# Autodesk Inventor assembly: B Drive
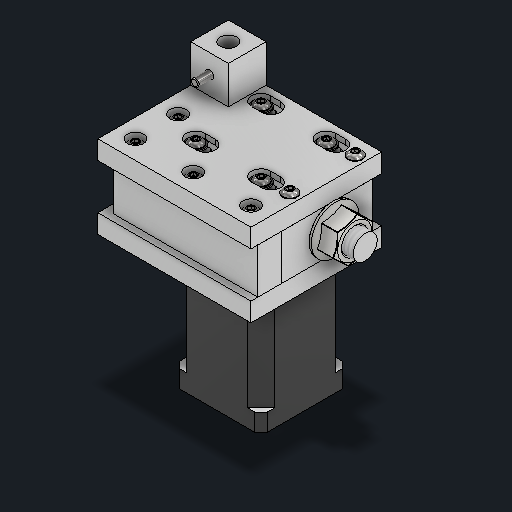
[picture p0: Inventor's stored thumbnail of the model, 512x512]
Saved by Autodesk Inventor 2025.1 (Build 291241020, 241B)
## iProperties
Created: 2025-05-09
Part Number: B Drive
Document SubType Name: Assembly
Designer: AdminForWorker
Title: B Drive
Author: AdminForWorker
## Documents named in this file (10)
- C:\Users\Joshua Eah\Documents\Voron 0.2\CAD\Master Assembly\Motion\AB Drives\Drives\B Drive.iam
- C:\Users\Joshua Eah\Documents\Voron 0.2\CAD\Machined Parts\AB Drives\B Drive\B Drive Assembly.iam
- C:\Users\Joshua Eah\Documents\Voron 0.2\CAD\Master Assembly\Hardware\M3x10 BHCS.ipt
- C:\Users\Joshua Eah\Documents\Voron 0.2\CAD\Master Assembly\Hardware\M3x35 BHCS.ipt
- C:\Users\Joshua Eah\Documents\Voron 0.2\CAD\Master Assembly\Hardware\M3x30 BHCS.ipt
- C:\Users\Joshua Eah\Documents\Voron 0.2\CAD\Master Assembly\Hardware\F623 Stack.iam
- C:\Users\Joshua Eah\Documents\Voron 0.2\CAD\Master Assembly\Hardware\M3 Hexnut.ipt
- C:\Users\Joshua Eah\Documents\Voron 0.2\CAD\Master Assembly\Hardware\M3_Washer.ipt
- C:\Users\Joshua Eah\Documents\Voron 0.2\CAD\Master Assembly\Motion\AB Drives\Motor Assembly\GT2 20T 6mm Pulley.iam
- C:\Users\Joshua Eah\Documents\Voron 0.2\CAD\Master Assembly\Motion\AB Drives\Motor Assembly\Nema14.ipt
## Components (26 placed, 9 different names)
1. B Drive Assembly:1 [sub-assembly] — Insert:4, Insert:5, Insert:10, Insert:11, Insert:12, Insert:13, Mate:5
2. GT2 20T 6mm Pulley:1 [sub-assembly] — Mate:1, Mate:2
3. Nema14:1 — Mate:1, Mate:2, Mate:3, Mate:4, Mate:5
4. M3x10 BHCS:1
5. M3x35 BHCS:1 — Insert:9, Mate:3
6. M3x35 BHCS:2
7. M3x35 BHCS:3
8. M3x35 BHCS:4
9. M3x35 BHCS:5 — Insert:7, Mate:4
10. M3x35 BHCS:6
11. M3x35 BHCS:7 — Insert:8
12. M3x35 BHCS:8 — Insert:6
13. M3x35 BHCS:9 — Insert:3, Insert:4
14. M3x30 BHCS:1
15. M3x30 BHCS:2 — Insert:5
16. M3 Hexnut:1
17. M3 Hexnut:2
18. M3 Hexnut:3
19. M3 Hexnut:4 — Insert:3
20. M3 Washer:1 — Insert:9, Insert:12
21. M3 Washer:2 — Insert:6, Insert:11
22. M3 Washer:3 — Insert:8, Insert:13
23. M3 Washer:4 — Insert:7, Insert:10
24. F623 Stack:1 [sub-assembly]
25. F623 Stack:2 [sub-assembly]
26. F623 Stack:3 [sub-assembly]
## Relationships (18: Insert 13, Mate 5)
- [Insert]: B Drive Assembly:1 ↔ M3x10 BHCS:1
- [Insert]: B Drive Assembly:1 ↔ M3x35 BHCS:6
- Insert:3: M3x35 BHCS:9 ↔ M3 Hexnut:4
- Insert:4: B Drive Assembly:1 ↔ M3x35 BHCS:9
- Insert:5: B Drive Assembly:1 ↔ M3x30 BHCS:2
- Insert:6: M3x35 BHCS:8 ↔ M3 Washer:2
- Insert:7: M3x35 BHCS:5 ↔ M3 Washer:4
- Insert:8: M3x35 BHCS:7 ↔ M3 Washer:3
- Insert:9: M3x35 BHCS:1 ↔ M3 Washer:1
- Insert:10: B Drive Assembly:1 ↔ M3 Washer:4
- Insert:11: B Drive Assembly:1 ↔ M3 Washer:2
- Insert:12: B Drive Assembly:1 ↔ M3 Washer:1
- Insert:13: B Drive Assembly:1 ↔ M3 Washer:3
- Mate:1: GT2 20T 6mm Pulley:1 ↔ Nema14:1
- Mate:2 (5.35 mm): GT2 20T 6mm Pulley:1 ↔ Nema14:1
- Mate:3: Nema14:1 ↔ M3x35 BHCS:1
- Mate:4: Nema14:1 ↔ M3x35 BHCS:5
- Mate:5: B Drive Assembly:1 ↔ Nema14:1
